# Autodesk Inventor assembly: Rubik's V2 assembly
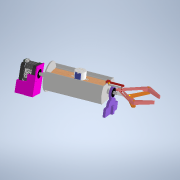
[picture p0: Inventor's stored thumbnail of the model, 180x180]
Saved by Autodesk Inventor 2020 (Build 240168000, 168)
## iProperties
Created: 2021-06-18
Part Number: Rubik's V2 assembly
Document SubType Name: Assembly
Designer: ugwue
Author: ugwue
## Documents named in this file (14)
- C:\Users\ugwue\OneDrive\Documents\rubik's cube\Rubik's V2 assembly.iam
- C:\Users\ugwue\OneDrive\Documents\rubik's cube\Casing.ipt
- C:\Users\ugwue\OneDrive\Documents\rubik's cube\Linear pinion.ipt
- C:\Users\ugwue\OneDrive\Documents\rubik's cube\Rack Base.ipt
- C:\Users\ugwue\OneDrive\Documents\rubik's cube\Rack.ipt
- C:\Users\ugwue\OneDrive\Documents\rubik's cube\28byj-48-5.snapshot.2\28BYJ-48 v5.iam
- C:\Users\ugwue\OneDrive\Documents\rubik's cube\Sliding linkage - V2.ipt
- C:\Users\ugwue\OneDrive\Documents\rubik's cube\Gripper Base V2.ipt
- C:\Users\ugwue\OneDrive\Documents\rubik's cube\Casing Cover.ipt
- C:\Users\ugwue\OneDrive\Documents\rubik's cube\Ball bearing.ipt
- C:\Users\ugwue\OneDrive\Documents\rubik's cube\Motor mount.ipt
- C:\Users\ugwue\OneDrive\Documents\rubik's cube\Secondary mount.ipt
- C:\Users\ugwue\OneDrive\Documents\rubik's cube\nema-17-step-motor-usongshine-17hs4401s-1.snapshot.2\Step - Nema 17 - 17HS4401S - Usongshine.ipt
- C:\Users\ugwue\OneDrive\Documents\rubik's cube\Grip Stopper.ipt
## Components (15 placed, 13 different names)
1. Casing:1 — Mate:2, Flush:5, Mate:3, Mate:4, Mate:5, Mate:6, Insert:6, Flush:11
2. Linear pinion:1 — Insert:1
3. Rack Base:1 — Mate:1, Flush:6, Flush:7, Flush:9, Mate:4, Mate:5, Mate:6, Flush:10
4. Rack:1 — Flush:7, Mate:7, Mate:8, Mate:9, Flush:10
5. 28BYJ-48 v5:1 [sub-assembly] — Mate:1, Insert:1, Flush:6, Flush:9
6. Sliding linkage - V2:1 — Insert:3, Tangent:1
7. Sliding linkage - V2:2 — Insert:2, Tangent:2
8. Gripper Base V2:1 — Insert:2, Insert:3, Mate:7, Mate:8, Mate:9
9. Casing Cover:1 — Mate:2, Flush:5, Mate:3, Insert:7, Mate:13, Mate:14
10. Ball bearing:1 — Insert:4, Insert:6
11. Motor mount:1 — Insert:4, Mate:10, Mate:11, Mate:12
12. Secondary mount:1 — Insert:5
13. Ball bearing:2 — Insert:5, Insert:7
14. Step - Nema 17 - 17HS4401S - Usongshine:1 — Mate:10, Mate:11, Mate:12
15. Grip Stopper:1 — Mate:13, Mate:14, Tangent:1, Tangent:2, Flush:11
## Relationships (29: Mate 14, Insert 7, Flush 6, Tangent 2)
- Mate:1: Rack Base:1 ↔ 28BYJ-48 v5:1
- Insert:1 (-5.5 mm): Linear pinion:1 ↔ 28BYJ-48 v5:1
- Insert:2 (-9 mm): Sliding linkage - V2:2 ↔ Gripper Base V2:1
- Insert:3 (-9 mm): Sliding linkage - V2:1 ↔ Gripper Base V2:1
- Mate:2: Casing:1 ↔ Casing Cover:1
- Flush:5: Casing:1 ↔ Casing Cover:1
- Mate:3: Casing:1 ↔ Casing Cover:1
- Flush:6 (26 mm): Rack Base:1 ↔ 28BYJ-48 v5:1
- Flush:7 (5 mm): Rack Base:1 ↔ Rack:1
- Flush:9 (65.5 mm): Rack Base:1 ↔ 28BYJ-48 v5:1
- Mate:4: Casing:1 ↔ Rack Base:1
- Mate:5: Casing:1 ↔ Rack Base:1
- Mate:6 (-4 mm): Casing:1 ↔ Rack Base:1
- Mate:7 (2.25 mm): Rack:1 ↔ Gripper Base V2:1
- Mate:8: Rack:1 ↔ Gripper Base V2:1
- Mate:9: Rack:1 ↔ Gripper Base V2:1
- Insert:4: Ball bearing:1 ↔ Motor mount:1
- Insert:5: Secondary mount:1 ↔ Ball bearing:2
- Insert:6 (-7 mm): Casing:1 ↔ Ball bearing:1
- Insert:7: Casing Cover:1 ↔ Ball bearing:2
- Mate:10: Motor mount:1 ↔ Step - Nema 17 - 17HS4401S - Usongshine:1
- Mate:11: Motor mount:1 ↔ Step - Nema 17 - 17HS4401S - Usongshine:1
- Mate:12: Motor mount:1 ↔ Step - Nema 17 - 17HS4401S - Usongshine:1
- Flush:10 (-1 mm): Rack Base:1 ↔ Rack:1
- Mate:13: Casing Cover:1 ↔ Grip Stopper:1
- Mate:14: Casing Cover:1 ↔ Grip Stopper:1
- Tangent:1: Sliding linkage - V2:1 ↔ Grip Stopper:1
- Tangent:2: Sliding linkage - V2:2 ↔ Grip Stopper:1
- Flush:11 (-33.5 mm): Casing:1 ↔ Grip Stopper:1
